# Autodesk Inventor assembly: 6 Plaction with hub and double pulley
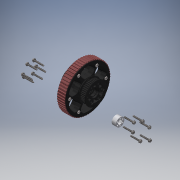
[picture p0: Inventor's stored thumbnail of the model, 180x180]
Saved by Autodesk Inventor 2018 (Build 220112000, 112)
## iProperties
Created: 2020-01-18
Part Number: 6 Plaction with hub and double pulley
Document SubType Name: Assembly
Designer: maste
Author: maste
Revision Number: ANY
## Documents named in this file (6)
- \\studenthome\students\S-2512711\GitHub\2020CAD\Drivebase AM14U1\Part Files\6 Plaction with hub and double pulley.iam
- \\studenthome\students\S-2512711\GitHub\2020CAD\Drivebase AM14U1\Part Files\42 tooth HTD Pulley half 2014.ipt
- \\studenthome\students\S-2512711\GitHub\2020CAD\Drivebase AM14U1\Part Files\10-24 Hex Washer Rolling x 1.25_93882A213.ipt
- \\studenthome\students\S-2512711\GitHub\2020CAD\Drivebase AM14U1\Part Files\500EX Hex Hub.ipt
- \\studenthome\students\S-2512711\GitHub\2020CAD\Drivebase AM14U1\Part Files\am-1305 500 Hex Spacer.ipt
- \\studenthome\students\S-2512711\GitHub\2020CAD\Gabriel Inventor Files (Shooter, Drivebase)\Drivebase Assembly\Part Files\am-3316 6 inch Plaction Wheel with Roughtop.iam
## Components (19 placed, 19 different names)
1. 42 tooth HTD Pulley half 2014_18 — Mate:1, Mate:2, Mate:3, Mate:4, Mate:6
2. 42 tooth HTD Pulley half 2014_19 — Mate:1, Mate:2, Mate:3, Mate:5
3. 10-24 Hex Washer Rolling x 1.25_93882A213_20
4. 10-24 Hex Washer Rolling x 1.25_93882A213_21
5. 10-24 Hex Washer Rolling x 1.25_93882A213_22
6. 10-24 Hex Washer Rolling x 1.25_93882A213_23
7. 10-24 Hex Washer Rolling x 1.25_93882A213_24
8. 10-24 Hex Washer Rolling x 1.25_93882A213_25
9. 42 tooth HTD Pulley half 2014_26 — Mate:7, Mate:8, Mate:9, Mate:11, Mate:12, Mate:14
10. 42 tooth HTD Pulley half 2014_27 — Mate:7, Mate:8, Mate:9, Mate:10, Mate:13
11. 500EX Hex Hub_28 — Mate:11, Mate:12, Mate:14
12. 10-24 Hex Washer Rolling x 1.25_93882A213_29
13. 10-24 Hex Washer Rolling x 1.25_93882A213_30
14. 10-24 Hex Washer Rolling x 1.25_93882A213_31
15. 10-24 Hex Washer Rolling x 1.25_93882A213_32
16. 10-24 Hex Washer Rolling x 1.25_93882A213_33
17. 10-24 Hex Washer Rolling x 1.25_93882A213_34
18. am-1305 500 Hex Spacer_35
19. am-3316 6 inch Plaction Wheel with Roughtop:1 [sub-assembly] — Mate:4, Mate:5, Mate:6, Mate:10, Mate:13
## Relationships (14: Mate 14)
- Mate:1: 42 tooth HTD Pulley half 2014_18 ↔ 42 tooth HTD Pulley half 2014_19
- Mate:2: 42 tooth HTD Pulley half 2014_18 ↔ 42 tooth HTD Pulley half 2014_19
- Mate:3: 42 tooth HTD Pulley half 2014_18 ↔ 42 tooth HTD Pulley half 2014_19
- Mate:4: 42 tooth HTD Pulley half 2014_18 ↔ am-3316 6 inch Plaction Wheel with Roughtop:1
- Mate:5: 42 tooth HTD Pulley half 2014_19 ↔ am-3316 6 inch Plaction Wheel with Roughtop:1
- Mate:6: 42 tooth HTD Pulley half 2014_18 ↔ am-3316 6 inch Plaction Wheel with Roughtop:1
- Mate:7: 42 tooth HTD Pulley half 2014_26 ↔ 42 tooth HTD Pulley half 2014_27
- Mate:8: 42 tooth HTD Pulley half 2014_26 ↔ 42 tooth HTD Pulley half 2014_27
- Mate:9: 42 tooth HTD Pulley half 2014_26 ↔ 42 tooth HTD Pulley half 2014_27
- Mate:10: 42 tooth HTD Pulley half 2014_27 ↔ am-3316 6 inch Plaction Wheel with Roughtop:1
- Mate:11: 42 tooth HTD Pulley half 2014_26 ↔ 500EX Hex Hub_28
- Mate:12: 42 tooth HTD Pulley half 2014_26 ↔ 500EX Hex Hub_28
- Mate:13: 42 tooth HTD Pulley half 2014_27 ↔ am-3316 6 inch Plaction Wheel with Roughtop:1
- Mate:14: 42 tooth HTD Pulley half 2014_26 ↔ 500EX Hex Hub_28
